# Autodesk Inventor assembly: nozzle
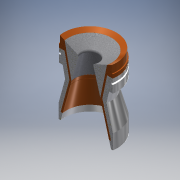
[picture p0: Inventor's stored thumbnail of the model, 180x180]
Saved by Autodesk Inventor 2017 SP1 (Build 210196100, 196)
## iProperties
Created: 2016-10-23
Part Number: nozzle
Document SubType Name: Assembly
Designer: cflannery
Author: cflannery
## Documents named in this file (6)
- D:\Triton_Rocket_Club\NONGIT\Nozzle_designSpace\nozzle.iam
- D:\Triton_Rocket_Club\NONGIT\Nozzle_designSpace\aluminum.ipt
- D:\Triton_Rocket_Club\NONGIT\Nozzle_designSpace\aluminum_retainer.ipt
- D:\Triton_Rocket_Club\NONGIT\Nozzle_designSpace\graphite.ipt
- D:\Triton_Rocket_Club\NONGIT\Nozzle_designSpace\phenolic_bottom.ipt
- D:\Triton_Rocket_Club\NONGIT\Nozzle_designSpace\phenolic_top.ipt
## Components (5 placed, 5 different names)
1. aluminum:1 — Mate:2, Mate:3, Mate:5, Mate:8
2. aluminum_retainer:1 — Mate:3, Mate:8
3. graphite:1 — Mate:1, Mate:4, Mate:6
4. phenolic_bottom:1 — Mate:1, Mate:2, Mate:7
5. phenolic_top:1 — Mate:4, Mate:5, Mate:6, Mate:7
## Relationships (8: Mate 8)
- Mate:1: graphite:1 ↔ phenolic_bottom:1
- Mate:2: aluminum:1 ↔ phenolic_bottom:1
- Mate:3: aluminum:1 ↔ aluminum_retainer:1
- Mate:4: graphite:1 ↔ phenolic_top:1
- Mate:5: aluminum:1 ↔ phenolic_top:1
- Mate:6: graphite:1 ↔ phenolic_top:1
- Mate:7: phenolic_bottom:1 ↔ phenolic_top:1
- Mate:8: aluminum:1 ↔ aluminum_retainer:1
